# Autodesk Inventor assembly: 6P Sprocket
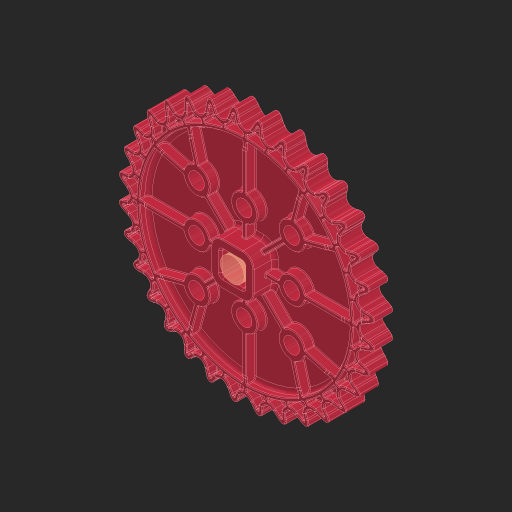
[picture p0: Inventor's stored thumbnail of the model, 512x512]
Saved by Autodesk Inventor 2023 (Build 270158000, 158)
## iProperties
Created: 2022-08-02
Part Number: 6P Sprocket
Document SubType Name: Assembly
Designer: ylu12
Author: ylu12
## Documents named in this file (3)
- C:\Users\ylu12\Documents\GitHub\VEX-CAD-Inventor\Motion\Sprockets\6P Sprocket\6P 32T Sprocket, No Insert.iam
- C:\Users\ylu12\Documents\GitHub\VEX-CAD-Inventor\Motion\Sprockets\Reference Files\6P 32T Sprocket.ipt
- C:\Users\ylu12\Documents\GitHub\VEX-CAD-Inventor\Motion\Sprockets\6P Sprocket.iam
## Components (1 placed, 1 different names)
1. 32T — Flush:6, Mate:11, Mate:12
## Relationships (3: Mate 2, Flush 1)
- Flush:6: 32T
- Mate:11: 32T
- Mate:12: 32T
